# Autodesk Inventor assembly: ResGalvoWobbleAssembly
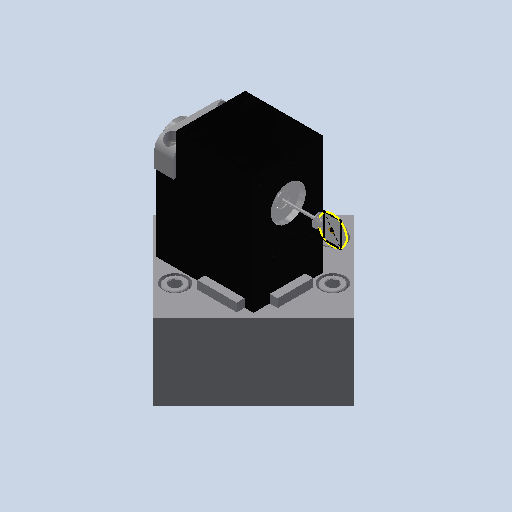
[picture p0: Inventor's stored thumbnail of the model, 512x512]
Saved by Autodesk Inventor 2022 (Build 260153000, 153)
## iProperties
Created: 2018-06-06
Part Number: ResGalvoWobbleAssembly
Document SubType Name: Assembly
Designer: legant_local
Author: legant_local
## Documents named in this file (11)
- G:\My Drive\2P-OPM\2P-OPM_CAD\workspace\Sub-assemblies\ResGalvoWobbleAssembly.iam
- G:\My Drive\2P-OPM\2P-OPM_CAD\workspace\Imported Components\Cambridge_Technology\CRS04K-S3-S-045 CRS 4kHz.ipt
- G:\My Drive\2P-OPM\2P-OPM_CAD\workspace\Imported Components\McMaster_Carr\McMaster_Carr_91585A351_dowel_pin_D3mm_L10mm.ipt
- G:\My Drive\2P-OPM\2P-OPM_CAD\workspace\Custom Parts Linked With Drawings\Thorlabs_20-1531-001_ResGalvoClamp.ipt
- G:\My Drive\2P-OPM\2P-OPM_CAD\workspace\Imported Components\Edmund\Edmund_36997_D25mm_T1mm_VISNIR_Window.ipt
- G:\My Drive\2P-OPM\2P-OPM_CAD\workspace\Imported Components\McMaster_Carr\McMaster_Carr_92290A747_M2x20mm_socket_cap.ipt
- G:\My Drive\2P-OPM\2P-OPM_CAD\workspace\Imported Components\McMaster_Carr\McMaster_Carr_92290A115_M3x10mm_socket_cap.ipt
- G:\My Drive\2P-OPM\2P-OPM_CAD\workspace\Custom Parts Linked With Drawings\ResGalvoWindow.ipt
- G:\My Drive\2P-OPM\2P-OPM_CAD\workspace\Custom Parts Linked With Drawings\ResGalvoMount_wobble.ipt
- G:\My Drive\2P-OPM\2P-OPM_CAD\workspace\Custom Parts Linked With Drawings\ResGalvoMount_base_plate.ipt
- G:\My Drive\2P-OPM\2P-OPM_CAD\workspace\Imported Components\McMaster_Carr\McMaster_Carr_92185A546_0.25in-20x1.5in_socket_cap.ipt
## Components (22 placed, 10 different names)
1. CRS04K-S3-S-045 CRS 4kHz:1 — Flush:1, Angle:1, Mate:31, Mate:32, Angle:3
2. ResGalvoMount_wobble:1 — Flush:1, Angle:1, Mate:2, Flush:2, Flush:3, Mate:3, Mate:4, Flush:4, Flush:5, Mate:5, Flush:6, Mate:7, Mate:8, Flush:7, Mate:13, Mate:14, Mate:15, Mate:16, Mate:17, Mate:18, Mate:19, Mate:20, Mate:21, Mate:22, Mate:23, Mate:24, Mate:31, Mate:32, Angle:3, Angle:4, Angle:5, Mate:35
3. ResGalvoWindow:1 — Mate:2, Flush:2, Flush:3, Mate:9, Mate:10, Mate:11, Mate:12
4. McMaster_Carr_91585A351_dowel_pin_D3mm_L10mm:1 — Mate:4, Flush:4
5. McMaster_Carr_91585A351_dowel_pin_D3mm_L10mm:2 — Mate:3, Flush:5
6. McMaster_Carr_91585A351_dowel_pin_D3mm_L10mm:3 — Mate:5, Flush:6
7. Thorlabs_20-1531-001_ResGalvoClamp:1 — Mate:7, Mate:8, Flush:7, Mate:25, Mate:26, Mate:27, Mate:28
8. Edmund_36997_D25mm_T1mm_VISNIR_Window:1 — Mate:9, Mate:10
9. Edmund_36997_D25mm_T1mm_VISNIR_Window:2 — Mate:11, Mate:12
10. McMaster_Carr_92290A747_M2x20mm_socket_cap:1 — Mate:13, Mate:14
11. McMaster_Carr_92290A747_M2x20mm_socket_cap:2 — Mate:15, Mate:20, Mate:33
12. McMaster_Carr_92290A747_M2x20mm_socket_cap:3 — Mate:16, Mate:19, Mate:34
13. McMaster_Carr_92290A747_M2x20mm_socket_cap:4 — Mate:17, Mate:18
14. McMaster_Carr_92290A747_M2x20mm_socket_cap:5 — Mate:21, Mate:24
15. McMaster_Carr_92290A747_M2x20mm_socket_cap:6 — Mate:22, Mate:23
16. McMaster_Carr_92290A115_M3x10mm_socket_cap:1 — Mate:25, Mate:26
17. McMaster_Carr_92290A115_M3x10mm_socket_cap:2 — Mate:27, Mate:28
18. ResGalvoMount_base_plate:1 — Angle:4, Angle:5, Mate:33, Mate:34, Mate:35, Mate:36, Mate:37, Mate:38, Mate:39, Mate:40, Mate:41, Mate:42, Mate:43
19. McMaster_Carr_92185A546_0.25in-20x1.5in_socket_cap:1 — Mate:39, Mate:43
20. McMaster_Carr_92185A546_0.25in-20x1.5in_socket_cap:2 — Mate:38, Mate:40
21. McMaster_Carr_92185A546_0.25in-20x1.5in_socket_cap:3 — Mate:36, Mate:42
22. McMaster_Carr_92185A546_0.25in-20x1.5in_socket_cap:4 — Mate:37, Mate:41
## Relationships (50: Mate 39, Flush 7, Angle 4)
- Flush:1 (-7 mm): CRS04K-S3-S-045 CRS 4kHz:1 ↔ ResGalvoMount_wobble:1
- Angle:1 (-45 deg): CRS04K-S3-S-045 CRS 4kHz:1 ↔ ResGalvoMount_wobble:1
- Mate:2: ResGalvoMount_wobble:1 ↔ ResGalvoWindow:1
- Flush:2: ResGalvoMount_wobble:1 ↔ ResGalvoWindow:1
- Flush:3: ResGalvoMount_wobble:1 ↔ ResGalvoWindow:1
- Mate:3: ResGalvoMount_wobble:1 ↔ McMaster_Carr_91585A351_dowel_pin_D3mm_L10mm:2
- Mate:4: ResGalvoMount_wobble:1 ↔ McMaster_Carr_91585A351_dowel_pin_D3mm_L10mm:1
- Flush:4 (-5 mm): ResGalvoMount_wobble:1 ↔ McMaster_Carr_91585A351_dowel_pin_D3mm_L10mm:1
- Flush:5 (-5 mm): ResGalvoMount_wobble:1 ↔ McMaster_Carr_91585A351_dowel_pin_D3mm_L10mm:2
- Mate:5: ResGalvoMount_wobble:1 ↔ McMaster_Carr_91585A351_dowel_pin_D3mm_L10mm:3
- Flush:6 (-5 mm): ResGalvoMount_wobble:1 ↔ McMaster_Carr_91585A351_dowel_pin_D3mm_L10mm:3
- Mate:7: ResGalvoMount_wobble:1 ↔ Thorlabs_20-1531-001_ResGalvoClamp:1
- Mate:8: ResGalvoMount_wobble:1 ↔ Thorlabs_20-1531-001_ResGalvoClamp:1
- Flush:7: ResGalvoMount_wobble:1 ↔ Thorlabs_20-1531-001_ResGalvoClamp:1
- Mate:9: ResGalvoWindow:1 ↔ Edmund_36997_D25mm_T1mm_VISNIR_Window:1
- Mate:10: ResGalvoWindow:1 ↔ Edmund_36997_D25mm_T1mm_VISNIR_Window:1
- Mate:11: ResGalvoWindow:1 ↔ Edmund_36997_D25mm_T1mm_VISNIR_Window:2
- Mate:12: ResGalvoWindow:1 ↔ Edmund_36997_D25mm_T1mm_VISNIR_Window:2
- Mate:13: ResGalvoMount_wobble:1 ↔ McMaster_Carr_92290A747_M2x20mm_socket_cap:1
- Mate:14: ResGalvoMount_wobble:1 ↔ McMaster_Carr_92290A747_M2x20mm_socket_cap:1
- Mate:15: ResGalvoMount_wobble:1 ↔ McMaster_Carr_92290A747_M2x20mm_socket_cap:2
- Mate:16: ResGalvoMount_wobble:1 ↔ McMaster_Carr_92290A747_M2x20mm_socket_cap:3
- Mate:17: ResGalvoMount_wobble:1 ↔ McMaster_Carr_92290A747_M2x20mm_socket_cap:4
- Mate:18: ResGalvoMount_wobble:1 ↔ McMaster_Carr_92290A747_M2x20mm_socket_cap:4
- Mate:19: ResGalvoMount_wobble:1 ↔ McMaster_Carr_92290A747_M2x20mm_socket_cap:3
- Mate:20: ResGalvoMount_wobble:1 ↔ McMaster_Carr_92290A747_M2x20mm_socket_cap:2
- Mate:21: ResGalvoMount_wobble:1 ↔ McMaster_Carr_92290A747_M2x20mm_socket_cap:5
- Mate:22: ResGalvoMount_wobble:1 ↔ McMaster_Carr_92290A747_M2x20mm_socket_cap:6
- Mate:23: ResGalvoMount_wobble:1 ↔ McMaster_Carr_92290A747_M2x20mm_socket_cap:6
- Mate:24: ResGalvoMount_wobble:1 ↔ McMaster_Carr_92290A747_M2x20mm_socket_cap:5
- Mate:25: Thorlabs_20-1531-001_ResGalvoClamp:1 ↔ McMaster_Carr_92290A115_M3x10mm_socket_cap:1
- Mate:26: Thorlabs_20-1531-001_ResGalvoClamp:1 ↔ McMaster_Carr_92290A115_M3x10mm_socket_cap:1
- Mate:27: Thorlabs_20-1531-001_ResGalvoClamp:1 ↔ McMaster_Carr_92290A115_M3x10mm_socket_cap:2
- Mate:28: Thorlabs_20-1531-001_ResGalvoClamp:1 ↔ McMaster_Carr_92290A115_M3x10mm_socket_cap:2
- Mate:31 (-35 mm): CRS04K-S3-S-045 CRS 4kHz:1 ↔ ResGalvoMount_wobble:1
- Mate:32: CRS04K-S3-S-045 CRS 4kHz:1 ↔ ResGalvoMount_wobble:1
- Angle:3 (0 deg): CRS04K-S3-S-045 CRS 4kHz:1 ↔ ResGalvoMount_wobble:1
- Angle:4 (0 deg): ResGalvoMount_wobble:1 ↔ ResGalvoMount_base_plate:1
- Angle:5 (45 deg): ResGalvoMount_wobble:1 ↔ ResGalvoMount_base_plate:1
- Mate:33: McMaster_Carr_92290A747_M2x20mm_socket_cap:2 ↔ ResGalvoMount_base_plate:1
- Mate:34: McMaster_Carr_92290A747_M2x20mm_socket_cap:3 ↔ ResGalvoMount_base_plate:1
- Mate:35: ResGalvoMount_wobble:1 ↔ ResGalvoMount_base_plate:1
- Mate:36: ResGalvoMount_base_plate:1 ↔ McMaster_Carr_92185A546_0.25in-20x1.5in_socket_cap:3
- Mate:37: ResGalvoMount_base_plate:1 ↔ McMaster_Carr_92185A546_0.25in-20x1.5in_socket_cap:4
- Mate:38: ResGalvoMount_base_plate:1 ↔ McMaster_Carr_92185A546_0.25in-20x1.5in_socket_cap:2
- Mate:39: ResGalvoMount_base_plate:1 ↔ McMaster_Carr_92185A546_0.25in-20x1.5in_socket_cap:1
- Mate:40: ResGalvoMount_base_plate:1 ↔ McMaster_Carr_92185A546_0.25in-20x1.5in_socket_cap:2
- Mate:41: ResGalvoMount_base_plate:1 ↔ McMaster_Carr_92185A546_0.25in-20x1.5in_socket_cap:4
- Mate:42: ResGalvoMount_base_plate:1 ↔ McMaster_Carr_92185A546_0.25in-20x1.5in_socket_cap:3
- Mate:43: ResGalvoMount_base_plate:1 ↔ McMaster_Carr_92185A546_0.25in-20x1.5in_socket_cap:1
